# Autodesk Inventor assembly: Right Rear Wheel with hub inside
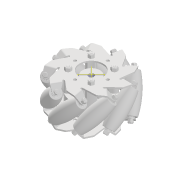
[picture p0: Inventor's stored thumbnail of the model, 180x180]
Saved by Autodesk Inventor 2020 (Build 240168000, 168)
## iProperties
Created: 2020-02-22
Part Number: Right Rear Wheel with hub inside
Document SubType Name: Assembly
Designer: ball
Author: ball
## Documents named in this file (5)
- C:\FTC\FTC8863CAD\2019 Robot\Mecanum Drive Train Metal\Right Rear Wheel with hub inside.iam
- C:\FTC\FTC8863CAD\GoBilda\1310 Parts\1310-0016-4008 assembly.ipt
- C:\FTC\FTC8863CAD\StepLibraries\Screws\M4 x 22 SOCKET HEAD CAP SCREW.ipt
- C:\FTC\FTC8863CAD\StepLibraries\Washers\M4 FLAT WASHER.ipt
- C:\FTC\FTC8863CAD\GoBilda\3213 Parts\3606-0000-0100 assembly.iam
## Components (10 placed, 4 different names)
1. 3606-0000-0100 assembly:1 [sub-assembly] — Mate:26, Mate:27, Mate:28, Mate:29, Mate:30, Mate:31, Mate:40, Mate:41, Mate:42, Mate:43, Mate:45, Mate:46
2. M4 x 22 SOCKET HEAD CAP SCREW:6 — Mate:31
3. M4 FLAT WASHER:6 — Mate:30
4. 1310-0016-4008 assembly:2 — Mate:26, Mate:27, Mate:28, Mate:29
5. M4 x 22 SOCKET HEAD CAP SCREW:7 — Mate:43
6. M4 FLAT WASHER:7 — Mate:40
7. M4 x 22 SOCKET HEAD CAP SCREW:8 — Mate:46
8. M4 FLAT WASHER:8 — Mate:42
9. M4 x 22 SOCKET HEAD CAP SCREW:9 — Mate:45
10. M4 FLAT WASHER:9 — Mate:41
## Relationships (20: Mate 20)
- [Mate]: M4 x 22 SOCKET HEAD CAP SCREW:6 ↔ M4 FLAT WASHER:6
- [Mate]: M4 x 22 SOCKET HEAD CAP SCREW:6 ↔ M4 FLAT WASHER:6
- Mate:26: 3606-0000-0100 assembly:1 ↔ 1310-0016-4008 assembly:2
- Mate:27: 3606-0000-0100 assembly:1 ↔ 1310-0016-4008 assembly:2
- Mate:28: 3606-0000-0100 assembly:1 ↔ 1310-0016-4008 assembly:2
- Mate:29: 3606-0000-0100 assembly:1 ↔ 1310-0016-4008 assembly:2
- Mate:30: 3606-0000-0100 assembly:1 ↔ M4 FLAT WASHER:6
- Mate:31: 3606-0000-0100 assembly:1 ↔ M4 x 22 SOCKET HEAD CAP SCREW:6
- [Mate]: M4 x 22 SOCKET HEAD CAP SCREW:7 ↔ M4 FLAT WASHER:7
- [Mate]: M4 x 22 SOCKET HEAD CAP SCREW:7 ↔ M4 FLAT WASHER:7
- [Mate]: M4 x 22 SOCKET HEAD CAP SCREW:8 ↔ M4 FLAT WASHER:8
- [Mate]: M4 x 22 SOCKET HEAD CAP SCREW:8 ↔ M4 FLAT WASHER:8
- [Mate]: M4 x 22 SOCKET HEAD CAP SCREW:9 ↔ M4 FLAT WASHER:9
- [Mate]: M4 x 22 SOCKET HEAD CAP SCREW:9 ↔ M4 FLAT WASHER:9
- Mate:40: 3606-0000-0100 assembly:1 ↔ M4 FLAT WASHER:7
- Mate:41: 3606-0000-0100 assembly:1 ↔ M4 FLAT WASHER:9
- Mate:42: 3606-0000-0100 assembly:1 ↔ M4 FLAT WASHER:8
- Mate:43: 3606-0000-0100 assembly:1 ↔ M4 x 22 SOCKET HEAD CAP SCREW:7
- Mate:45: 3606-0000-0100 assembly:1 ↔ M4 x 22 SOCKET HEAD CAP SCREW:9
- Mate:46: 3606-0000-0100 assembly:1 ↔ M4 x 22 SOCKET HEAD CAP SCREW:8
## Named parameters: d56_d39_d14_d12 = 0 mm, d57_d40_d15_d13 = 0 mm, d64_d56_d39_d14_d12 = 0 mm, d65_d57_d40_d15_d13 = 0 mm, d66_d56_d39_d14_d12 = 0 mm, d67_d57_d40_d15_d13 = 0 mm, d68_d56_d39_d14_d12 = 0 mm, d69_d57_d40_d15_d13 = 0 mm
